# Autodesk Inventor assembly: EnsamblajE_BRAZO_Y_SUJECIONES
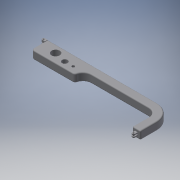
[picture p0: Inventor's stored thumbnail of the model, 180x180]
Saved by Autodesk Inventor 2019.4 (Build 234330000, 330)
## iProperties
Created: 2020-08-24
Part Number: EnsamblajE_BRAZO_Y_SUJECIONES
Document SubType Name: Assembly
Designer: crist
Author: crist
## Documents named in this file (3)
- C:\Users\crist\Desktop\BRAZO_UNDIMOTRIZ\EnsamblajE_BRAZO_Y_SUJECIONES.iam
- C:\Users\crist\Desktop\BALSA_UNDIMOTRIZ\SUJECION_BALSA_UNDIMOTRIZ.ipt
- C:\Users\crist\Desktop\BRAZO_UNDIMOTRIZ\BRAZO BALSA UNDIMOTRIZ.ipt
## Components (8 placed, 2 different names)
1. SUJECION_BALSA_UNDIMOTRIZ:3
2. SUJECION_BALSA_UNDIMOTRIZ:4 — Rígido:1
3. SUJECION_BALSA_UNDIMOTRIZ:5 — Rígido:7
4. SUJECION_BALSA_UNDIMOTRIZ:6
5. BRAZO BALSA UNDIMOTRIZ:1 — Rígido:1
6. SUJECION_BALSA_UNDIMOTRIZ:8 — Rígido:4
7. SUJECION_BALSA_UNDIMOTRIZ:9 — Rígido:4
8. SUJECION_BALSA_UNDIMOTRIZ:10 — Rígido:7
## Relationships (3: WeldJoint 3)
- Rígido:1 [WeldJoint]: SUJECION_BALSA_UNDIMOTRIZ:4 ↔ BRAZO BALSA UNDIMOTRIZ:1
- Rígido:4 [WeldJoint]: SUJECION_BALSA_UNDIMOTRIZ:8 ↔ SUJECION_BALSA_UNDIMOTRIZ:9
- Rígido:7 [WeldJoint]: SUJECION_BALSA_UNDIMOTRIZ:5 ↔ SUJECION_BALSA_UNDIMOTRIZ:10
